# Autodesk Inventor assembly: Track Assembly
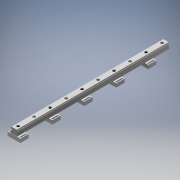
[picture p0: Inventor's stored thumbnail of the model, 180x180]
Saved by Autodesk Inventor 2016 (Build 200138000, 138)
## iProperties
Created: 2015-07-08
Part Number: Track Assembly
Document SubType Name: Assembly
Designer: Dennis
Author: Dennis
## Documents named in this file (4)
- C:\Users\Matthew Cheung\Dropbox\Work\National Instruments\Shared Folder\NI Ball Bearing Slider Crank\CAD\Assemblies\Track Assembly.iam
- C:\Users\Matthew Cheung\Dropbox\Work\National Instruments\Shared Folder\NI Ball Bearing Slider Crank\CAD\McMaster Parts\Ball Bearing Guide Rail - Guide Rail, 34mm Wide, for Ball-Bearing Carriage - 6709K702.ipt
- C:\Users\Matthew Cheung\Dropbox\Work\National Instruments\Shared Folder\NI Ball Bearing Slider Crank\CAD\Track Foot.ipt
- C:\Users\Matthew Cheung\Dropbox\Work\National Instruments\Shared Folder\NI Ball Bearing Slider Crank\CAD\McMaster Parts\M5x1.25x30.ipt
## Components (11 placed, 3 different names)
1. Ball Bearing Guide Rail - Guide Rail, 34mm Wide, for Ball-Bearing Carriage - 6709K702:1 — Mate:1, Mate:2, Mate:3, Mate:4, Mate:5, Mate:6, Mate:7, Mate:8, Mate:9, Mate:10, Mate:11, Mate:12, Mate:13, Mate:14, Mate:15, Mate:16, Mate:17, Mate:18, Mate:19, Mate:20
2. Track Foot:1 — Angle:1, Mate:1, Mate:2
3. Track Foot:2 — Angle:2, Mate:3, Mate:4
4. Track Foot:3 — Angle:3, Mate:5, Mate:6
5. Track Foot:4 — Angle:4, Mate:7, Mate:8
6. Track Foot:5 — Angle:5, Mate:9, Mate:10
7. M5x1.25x30:1 — Mate:11, Mate:16
8. M5x1.25x30:2 — Mate:12, Mate:17
9. M5x1.25x30:3 — Mate:13, Mate:18
10. M5x1.25x30:4 — Mate:14, Mate:19
11. M5x1.25x30:5 — Mate:15, Mate:20
## Relationships (25: Mate 20, Angle 5)
- Angle:1 (0 deg): Track Foot:1
- Mate:1: Ball Bearing Guide Rail - Guide Rail, 34mm Wide, for Ball-Bearing Carriage - 6709K702:1 ↔ Track Foot:1
- Mate:2: Ball Bearing Guide Rail - Guide Rail, 34mm Wide, for Ball-Bearing Carriage - 6709K702:1 ↔ Track Foot:1
- Angle:2 (0 deg): Track Foot:2
- Mate:3: Ball Bearing Guide Rail - Guide Rail, 34mm Wide, for Ball-Bearing Carriage - 6709K702:1 ↔ Track Foot:2
- Mate:4: Ball Bearing Guide Rail - Guide Rail, 34mm Wide, for Ball-Bearing Carriage - 6709K702:1 ↔ Track Foot:2
- Angle:3 (0 deg): Track Foot:3
- Mate:5: Ball Bearing Guide Rail - Guide Rail, 34mm Wide, for Ball-Bearing Carriage - 6709K702:1 ↔ Track Foot:3
- Mate:6: Ball Bearing Guide Rail - Guide Rail, 34mm Wide, for Ball-Bearing Carriage - 6709K702:1 ↔ Track Foot:3
- Angle:4 (0 deg): Track Foot:4
- Mate:7: Ball Bearing Guide Rail - Guide Rail, 34mm Wide, for Ball-Bearing Carriage - 6709K702:1 ↔ Track Foot:4
- Mate:8: Ball Bearing Guide Rail - Guide Rail, 34mm Wide, for Ball-Bearing Carriage - 6709K702:1 ↔ Track Foot:4
- Angle:5 (0 deg): Track Foot:5
- Mate:9: Ball Bearing Guide Rail - Guide Rail, 34mm Wide, for Ball-Bearing Carriage - 6709K702:1 ↔ Track Foot:5
- Mate:10: Ball Bearing Guide Rail - Guide Rail, 34mm Wide, for Ball-Bearing Carriage - 6709K702:1 ↔ Track Foot:5
- Mate:11: Ball Bearing Guide Rail - Guide Rail, 34mm Wide, for Ball-Bearing Carriage - 6709K702:1 ↔ M5x1.25x30:1
- Mate:12: Ball Bearing Guide Rail - Guide Rail, 34mm Wide, for Ball-Bearing Carriage - 6709K702:1 ↔ M5x1.25x30:2
- Mate:13: Ball Bearing Guide Rail - Guide Rail, 34mm Wide, for Ball-Bearing Carriage - 6709K702:1 ↔ M5x1.25x30:3
- Mate:14: Ball Bearing Guide Rail - Guide Rail, 34mm Wide, for Ball-Bearing Carriage - 6709K702:1 ↔ M5x1.25x30:4
- Mate:15: Ball Bearing Guide Rail - Guide Rail, 34mm Wide, for Ball-Bearing Carriage - 6709K702:1 ↔ M5x1.25x30:5
- Mate:16: Ball Bearing Guide Rail - Guide Rail, 34mm Wide, for Ball-Bearing Carriage - 6709K702:1 ↔ M5x1.25x30:1
- Mate:17: Ball Bearing Guide Rail - Guide Rail, 34mm Wide, for Ball-Bearing Carriage - 6709K702:1 ↔ M5x1.25x30:2
- Mate:18: Ball Bearing Guide Rail - Guide Rail, 34mm Wide, for Ball-Bearing Carriage - 6709K702:1 ↔ M5x1.25x30:3
- Mate:19: Ball Bearing Guide Rail - Guide Rail, 34mm Wide, for Ball-Bearing Carriage - 6709K702:1 ↔ M5x1.25x30:4
- Mate:20: Ball Bearing Guide Rail - Guide Rail, 34mm Wide, for Ball-Bearing Carriage - 6709K702:1 ↔ M5x1.25x30:5
